# Autodesk Inventor assembly: Arduino-Bot-Baugruppe
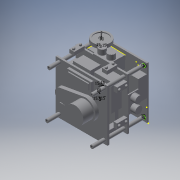
[picture p0: Inventor's stored thumbnail of the model, 180x180]
Saved by Autodesk Inventor 2019.5 (Build 235369000, 369)
## iProperties
Created: 2021-09-30
Part Number: Arduino-Bot-Baugruppe
Material: Generisch
Document SubType Name: Assembly
Designer: mritt
Author: mritt
## Documents named in this file (17)
- D:\Studium\Universität Stuttgart\Sonstige Tätigkeiten\Tätigkeit_studentische_Hilfskraft_Informatik\Hiwi-Projekt\CAD-Dateien\Arduino-Bot\Arduino-Bot-Baugruppe.iam
- D:\Studium\Universität Stuttgart\Sonstige Tätigkeiten\Tätigkeit_studentische_Hilfskraft_Informatik\Hiwi-Projekt\CAD-Dateien\Arduino-Bot\Grundplatte1.ipt
- D:\Studium\Universität Stuttgart\Sonstige Tätigkeiten\Tätigkeit_studentische_Hilfskraft_Informatik\Hiwi-Projekt\CAD-Dateien\Arduino-Bot\Grundplatte.ipt
- D:\Studium\Universität Stuttgart\Sonstige Tätigkeiten\Tätigkeit_studentische_Hilfskraft_Informatik\Hiwi-Projekt\CAD-Dateien\Arduino-Bot\Stangen.ipt
- D:\Studium\Universität Stuttgart\Sonstige Tätigkeiten\Tätigkeit_studentische_Hilfskraft_Informatik\Hiwi-Projekt\CAD-Dateien\Arduino-Bot\9V-Blockbaterie.ipt
- D:\Studium\Universität Stuttgart\Sonstige Tätigkeiten\Tätigkeit_studentische_Hilfskraft_Informatik\Hiwi-Projekt\CAD-Dateien\Arduino-Bot\Linien-Sensor.ipt
- D:\Studium\Universität Stuttgart\Sonstige Tätigkeiten\Tätigkeit_studentische_Hilfskraft_Informatik\Hiwi-Projekt\CAD-Dateien\Arduino-Bot\Motor_rechts.ipt
- D:\Studium\Universität Stuttgart\Sonstige Tätigkeiten\Tätigkeit_studentische_Hilfskraft_Informatik\Hiwi-Projekt\CAD-Dateien\Arduino-Bot\Motor_links.ipt
- D:\Studium\Universität Stuttgart\Sonstige Tätigkeiten\Tätigkeit_studentische_Hilfskraft_Informatik\Hiwi-Projekt\CAD-Dateien\Arduino-Bot\Ultraschallsensor.ipt
- D:\Studium\Universität Stuttgart\Sonstige Tätigkeiten\Tätigkeit_studentische_Hilfskraft_Informatik\Hiwi-Projekt\CAD-Dateien\Arduino-Bot\Battery-Controller.ipt
- D:\Studium\Universität Stuttgart\Sonstige Tätigkeiten\Tätigkeit_studentische_Hilfskraft_Informatik\Hiwi-Projekt\CAD-Dateien\Arduino-Bot\IR-Sensor.ipt
- D:\Studium\Universität Stuttgart\Sonstige Tätigkeiten\Tätigkeit_studentische_Hilfskraft_Informatik\Hiwi-Projekt\CAD-Dateien\Arduino-Bot\Arduino.ipt
- D:\Studium\Universität Stuttgart\Sonstige Tätigkeiten\Tätigkeit_studentische_Hilfskraft_Informatik\Hiwi-Projekt\CAD-Dateien\Arduino-Bot\Platiene-Arduino.ipt
- D:\Studium\Universität Stuttgart\Sonstige Tätigkeiten\Tätigkeit_studentische_Hilfskraft_Informatik\Hiwi-Projekt\CAD-Dateien\Arduino-Bot\Rad.ipt
- D:\Studium\Universität Stuttgart\Sonstige Tätigkeiten\Tätigkeit_studentische_Hilfskraft_Informatik\Hiwi-Projekt\CAD-Dateien\Arduino-Bot\LIDAR-Sensor.ipt
- D:\Studium\Universität Stuttgart\Sonstige Tätigkeiten\Tätigkeit_studentische_Hilfskraft_Informatik\Hiwi-Projekt\CAD-Dateien\Arduino-Bot\Wifi-Board.ipt
- D:\Studium\Universität Stuttgart\Sonstige Tätigkeiten\Tätigkeit_studentische_Hilfskraft_Informatik\Hiwi-Projekt\CAD-Dateien\Arduino-Bot\LCD-Display.ipt
## Components (32 placed, 16 different names)
1. Grundplatte1:1 — Passend:1, Passend:2, Passend:3, Passend:4, Passend:5, Passend:6, Passend:7, Passend:12, Passend:13, Passend:14, Passend:15, Passend:16, Fluchtend:4, Fluchtend:5, Passend:19, Fluchtend:6
2. Grundplatte:1 — Passend:8, Passend:9, Passend:10, Passend:11, Passend:18, Fluchtend:2, Fluchtend:3, Passend:20, Passend:21, Passend:22, Passend:23, Passend:24, Passend:25, Passend:26, Fluchtend:7, Fluchtend:8, Fluchtend:9, Fluchtend:10, Passend:27, Fluchtend:11, Fluchtend:12, Fluchtend:13, Fluchtend:14, Fluchtend:15, Passend:30, Passend:31, Passend:32, Fluchtend:16, Fluchtend:17, Fluchtend:18
3. Grundplatte:2 — Passend:28, Passend:29, Passend:35, Passend:36, Passend:37
4. Stangen:1 — Passend:1, Passend:9
5. Stangen:2 — Passend:2, Passend:6, Passend:11
6. Stangen:3 — Passend:3, Passend:7, Passend:8, Passend:29
7. Stangen:4 — Passend:4, Passend:5, Passend:10, Passend:28
8. 9V-Blockbaterie:1 — Passend:12, Fluchtend:4
9. Linien-Sensor:1 — Passend:13, Passend:14
10. Motor_rechts:1 — Passend:15, Passend:17, Fluchtend:1, Passend:33
11. Motor_links:1 — Passend:16, Passend:17, Fluchtend:1, Passend:34
12. Ultraschallsensor:1 — Passend:18, Fluchtend:2, Fluchtend:3
13. Battery-Controller:1 — Fluchtend:5, Passend:19, Fluchtend:6
14. Ultraschallsensor:2 — Passend:21, Fluchtend:8, Fluchtend:16
15. Ultraschallsensor:3 — Passend:20, Fluchtend:7, Fluchtend:18
16. Ultraschallsensor:4 — Passend:22, Fluchtend:9, Fluchtend:17
17. IR-Sensor:1 — Passend:23, Passend:24
18. IR-Sensor:2 — Passend:25, Passend:26
19. IR-Sensor:3 — Fluchtend:10, Passend:27
20. IR-Sensor:4 — Fluchtend:15
21. IR-Sensor:5 — Fluchtend:14
22. IR-Sensor:6 — Fluchtend:13
23. IR-Sensor:7 — Fluchtend:11
24. IR-Sensor:8 — Fluchtend:12
25. Arduino:1 — Passend:30
26. Arduino:2 — Passend:31
27. Platiene-Arduino:1 — Passend:32
28. Rad:1 — Passend:33
29. Rad:2 — Passend:34
30. LIDAR-Sensor:1 — Passend:35
31. Wifi-Board:1 — Passend:36
32. LCD-Display:1 — Passend:37
## Relationships (55: Mate 37, Flush 18)
- Passend:1 [Mate]: Grundplatte1:1 ↔ Stangen:1
- Passend:2 [Mate]: Grundplatte1:1 ↔ Stangen:2
- Passend:3 [Mate]: Grundplatte1:1 ↔ Stangen:3
- Passend:4 [Mate]: Grundplatte1:1 ↔ Stangen:4
- Passend:5 [Mate]: Grundplatte1:1 ↔ Stangen:4
- Passend:6 [Mate]: Grundplatte1:1 ↔ Stangen:2
- Passend:7 [Mate]: Grundplatte1:1 ↔ Stangen:3
- Passend:8 [Mate]: Grundplatte:1 ↔ Stangen:3
- Passend:9 [Mate]: Grundplatte:1 ↔ Stangen:1
- Passend:10 [Mate]: Grundplatte:1 ↔ Stangen:4
- Passend:11 [Mate]: Grundplatte:1 ↔ Stangen:2
- Passend:12 [Mate]: Grundplatte1:1 ↔ 9V-Blockbaterie:1
- Passend:13 [Mate]: Grundplatte1:1 ↔ Linien-Sensor:1
- Passend:14 [Mate]: Grundplatte1:1 ↔ Linien-Sensor:1
- Passend:15 [Mate]: Grundplatte1:1 ↔ Motor_rechts:1
- Passend:16 [Mate]: Grundplatte1:1 ↔ Motor_links:1
- Passend:17 [Mate] (63.5 mm): Motor_rechts:1 ↔ Motor_links:1
- Fluchtend:1 [Flush]: Motor_rechts:1 ↔ Motor_links:1
- Passend:18 [Mate]: Grundplatte:1 ↔ Ultraschallsensor:1
- Fluchtend:2 [Flush]: Grundplatte:1 ↔ Ultraschallsensor:1
- Fluchtend:3 [Flush] (-50 mm): Grundplatte:1 ↔ Ultraschallsensor:1
- Fluchtend:4 [Flush]: Grundplatte1:1 ↔ 9V-Blockbaterie:1
- Fluchtend:5 [Flush] (-50 mm): Grundplatte1:1 ↔ Battery-Controller:1
- Passend:19 [Mate]: Grundplatte1:1 ↔ Battery-Controller:1
- Fluchtend:6 [Flush] (-60 mm): Grundplatte1:1 ↔ Battery-Controller:1
- Passend:20 [Mate]: Grundplatte:1 ↔ Ultraschallsensor:3
- Passend:21 [Mate]: Grundplatte:1 ↔ Ultraschallsensor:2
- Passend:22 [Mate]: Grundplatte:1 ↔ Ultraschallsensor:4
- Passend:23 [Mate]: Grundplatte:1 ↔ IR-Sensor:1
- Passend:24 [Mate]: Grundplatte:1 ↔ IR-Sensor:1
- Passend:25 [Mate]: Grundplatte:1 ↔ IR-Sensor:2
- Passend:26 [Mate]: Grundplatte:1 ↔ IR-Sensor:2
- Fluchtend:7 [Flush]: Grundplatte:1 ↔ Ultraschallsensor:3
- Fluchtend:8 [Flush]: Grundplatte:1 ↔ Ultraschallsensor:2
- Fluchtend:9 [Flush]: Grundplatte:1 ↔ Ultraschallsensor:4
- Fluchtend:10 [Flush]: Grundplatte:1 ↔ IR-Sensor:3
- Passend:27 [Mate]: Grundplatte:1 ↔ IR-Sensor:3
- Fluchtend:11 [Flush]: Grundplatte:1 ↔ IR-Sensor:7
- Fluchtend:12 [Flush]: Grundplatte:1 ↔ IR-Sensor:8
- Fluchtend:13 [Flush]: Grundplatte:1 ↔ IR-Sensor:6
- Fluchtend:14 [Flush]: Grundplatte:1 ↔ IR-Sensor:5
- Fluchtend:15 [Flush]: Grundplatte:1 ↔ IR-Sensor:4
- Passend:28 [Mate]: Grundplatte:2 ↔ Stangen:4
- Passend:29 [Mate]: Grundplatte:2 ↔ Stangen:3
- Passend:30 [Mate]: Grundplatte:1 ↔ Arduino:1
- Passend:31 [Mate]: Grundplatte:1 ↔ Arduino:2
- Passend:32 [Mate]: Grundplatte:1 ↔ Platiene-Arduino:1
- Passend:33 [Mate]: Motor_rechts:1 ↔ Rad:1
- Passend:34 [Mate]: Motor_links:1 ↔ Rad:2
- Fluchtend:16 [Flush] (-50 mm): Grundplatte:1 ↔ Ultraschallsensor:2
- Fluchtend:17 [Flush] (-50 mm): Grundplatte:1 ↔ Ultraschallsensor:4
- Fluchtend:18 [Flush] (-50 mm): Grundplatte:1 ↔ Ultraschallsensor:3
- Passend:35 [Mate]: Grundplatte:2 ↔ LIDAR-Sensor:1
- Passend:36 [Mate]: Grundplatte:2 ↔ Wifi-Board:1
- Passend:37 [Mate]: Grundplatte:2 ↔ LCD-Display:1
